# Autodesk Inventor assembly: ASY MSC 900.4  base frame
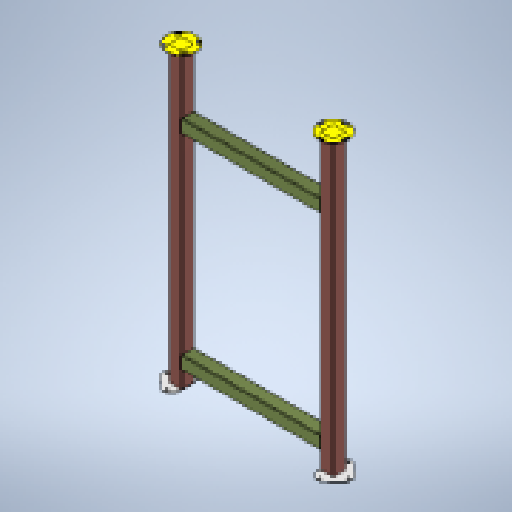
[picture p0: Inventor's stored thumbnail of the model, 512x512]
Saved by Autodesk Inventor 2025 (Build 290162010, 162A)
## iProperties
_SolveAssemblyDoc: Frame Generator Solve Assembly
_Version: 25.0.0
Created: 2024-06-30
Part Number: ASY MSC 900.4  base frame
Document SubType Name: Assembly
Designer: pokla
Stock Number: ASY МОО 900.4 базовая рама
Author: pokla
## Documents named in this file (5)
- C:\Users\user\YandexDisk\домашниий пк\Inventor\Manturovo\Manturovo_Se-clar\ASY MSC 120.1  base frame.iam
- C:\Users\user\YandexDisk\домашниий пк\Inventor\Manturovo\Manturovo_Se-clar\ASY MSC 120.1  base frame.ipt
- C:\Users\user\YandexDisk\домашниий пк\Inventor\Manturovo\Manturovo_Se-clar\ASY MSC 120.1  base frame\Frame\Frame 1719748116978.iam
- C:\Users\user\YandexDisk\домашниий пк\Inventor\Manturovo\Manturovo_Se-clar\MSC 127 flange frame heel.ipt
- C:\Users\user\YandexDisk\домашниий пк\Inventor\Manturovo\Manturovo_Se-clar\MSC 126 flange frame.ipt
## Components (6 placed, 4 different names)
1. ASY MSC 120.1  base frame.ipt:1
2. Frame 1719748116978.iam:1 [sub-assembly] — Rigid:3, Rigid:4, Rigid:5, Rigid:6
3. MSC 127 flange frame heel.ipt:1 — Rigid:6
4. MSC 127 flange frame heel.ipt:2 — Rigid:5
5. MSC 126 flange frame.ipt:1 — Rigid:3
6. MSC 126 flange frame.ipt:2 — Rigid:4
## Relationships (4: WeldJoint 4)
- Rigid:3 [WeldJoint]: Frame 1719748116978.iam:1 ↔ MSC 126 flange frame.ipt:1
- Rigid:4 [WeldJoint]: Frame 1719748116978.iam:1 ↔ MSC 126 flange frame.ipt:2
- Rigid:5 [WeldJoint]: Frame 1719748116978.iam:1 ↔ MSC 127 flange frame heel.ipt:2
- Rigid:6 [WeldJoint]: Frame 1719748116978.iam:1 ↔ MSC 127 flange frame heel.ipt:1
